# Autodesk Inventor assembly: LowerBody
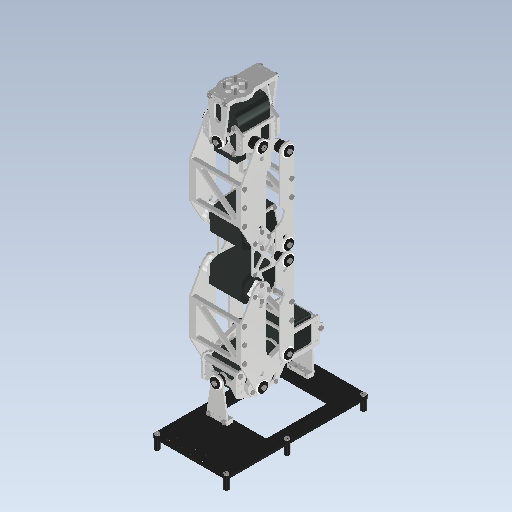
[picture p0: Inventor's stored thumbnail of the model, 512x512]
Saved by Autodesk Inventor 2020.4 (Build 244396010, 396A)
## iProperties
Created: 2021-10-01
Part Number: LowerBody
Document SubType Name: Assembly
Designer: Masato
Mass: 1009.03 g
Surface Area: 2721.67 cm^2
Volume: 456.516 cm^3
Density: 2.21029 g/cm^3
Author: Masato
## Documents named in this file (15)
- C:\Users\t-nagamine\Documents\Cit Brains\OpenPlatform_ver3_0\LowerBody\LowerBody.iam
- C:\Users\t-nagamine\Documents\Cit Brains\OpenPlatform_ver3_0\LowerBody\Ankle\Ankle.iam
- C:\Users\t-nagamine\Documents\Cit Brains\OpenPlatform_ver3_0\LowerBody\Ankle\Ankle_side_pitch.iam
- C:\Users\t-nagamine\Documents\Cit Brains\OpenPlatform_ver3_0\LowerBody\Foot\Foot.iam
- C:\Users\t-nagamine\Documents\Cit Brains\OpenPlatform_ver3_0\LowerBody\Knee\Knee.iam
- C:\Users\t-nagamine\Documents\Cit Brains\OpenPlatform_ver3_0\LowerBody\Leg_joit\Leg_joint_roll_pitch.iam
- C:\Users\t-nagamine\Documents\Cit Brains\OpenPlatform_ver3_0\LowerBody\Leg_joit\Leg_joint_roll_yaw.iam
- C:\Users\t-nagamine\Documents\Cit Brains\OpenPlatform_ver3_0\LowerBody\Slider_crank\Slider_crank_mechanism.iam
- C:\Users\t-nagamine\Documents\Cit Brains\OpenPlatform_ver3_0\LowerBody\Link\BackLink.iam
- C:\Users\t-nagamine\Documents\Cit Brains\OpenPlatform_ver3_0\LowerBody\Link\FrontLink.iam
- C:\Users\t-nagamine\Documents\Cit Brains\OpenPlatform_ver3_0\Ready_Made\Screw\M2_6-6.ipt
- C:\Users\t-nagamine\Documents\Cit Brains\OpenPlatform_ver3_0\Ready_Made\Screw\M3-6.ipt
- C:\Users\t-nagamine\Documents\Cit Brains\OpenPlatform_ver3_0\Ready_Made\Screw\M2_6-10.ipt
- C:\Users\t-nagamine\Documents\Cit Brains\OpenPlatform_ver3_0\Ready_Made\Screw\M3-8.ipt
- C:\Users\t-nagamine\Documents\Cit Brains\OpenPlatform_ver3_0\Ready_Made\Screw\M3-10.ipt
## Components (53 placed, 14 different names)
1. Ankle:1 [sub-assembly] — 挿入:15, 挿入:21, 挿入:22, 角度:11
2. Ankle_side_pitch:1 [sub-assembly] — 挿入:21, 挿入:23, 挿入:24, 挿入:25, 挿入:26, 挿入:35, 挿入:36, フラッシュ:5
3. Ankle_side_pitch:2 [sub-assembly] — 挿入:22, 挿入:27, 挿入:28, 挿入:29, 挿入:30, フラッシュ:5
4. Foot:1 [sub-assembly] — 挿入:15, 挿入:17, 挿入:18, 挿入:19, 挿入:20, 角度:3, 角度:5, 挿入:67
5. Knee:1 [sub-assembly] — 挿入:31, 挿入:32, 挿入:33, 挿入:34
6. Leg_joint_roll_pitch:1 [sub-assembly] — 挿入:2, 挿入:37, 挿入:38, 角度:6, 角度:9, 角度:10, 挿入:70
7. Leg_joint_roll_yaw:1 [sub-assembly] — メイト:1, フラッシュ:3, フラッシュ:4, 角度:5, 角度:6, 挿入:69, 挿入:70
8. Slider_crank_mechanism:1 [sub-assembly] — 挿入:2, 挿入:69
9. BackLink:1 [sub-assembly] — 挿入:33, 挿入:36, 挿入:42, 挿入:46, 挿入:64, 挿入:66, 角度:7
10. FrontLink:1 [sub-assembly] — 挿入:31, 挿入:35, 角度:3, 挿入:51, 挿入:52, 挿入:53, 挿入:54, 挿入:59, 挿入:60, 挿入:61, 挿入:62, 挿入:63, 挿入:65, 角度:7, 角度:11, 角度:12
11. BackLink:2 [sub-assembly] — 挿入:34, 挿入:38, 挿入:39, 挿入:41, 挿入:44, 挿入:45, 角度:8
12. FrontLink:2 [sub-assembly] — 挿入:32, 挿入:37, 挿入:40, 挿入:43, 挿入:47, 挿入:48, 挿入:49, 挿入:50, 挿入:55, 挿入:56, 挿入:57, 挿入:58, 角度:8, 角度:10, 角度:12, 角度:9
13. M2_6-6:9 — 挿入:17
14. M2_6-6:10 — 挿入:18
15. M2_6-6:11 — 挿入:19
16. M2_6-6:12 — 挿入:20
17. M2_6-6:13 — 挿入:23
18. M2_6-6:14 — 挿入:24
19. M2_6-6:15 — 挿入:25
20. M2_6-6:16 — 挿入:26
21. M2_6-6:17 — 挿入:27
22. M2_6-6:18 — 挿入:28
23. M2_6-6:19 — 挿入:29
24. M2_6-6:20 — 挿入:30
25. M3-6:4 — 挿入:40
26. M3-6:5 — 挿入:39
27. M3-6:6 — 挿入:44
28. M3-6:7 — 挿入:43
29. M3-6:8 — 挿入:41
30. M3-6:9 — 挿入:45
31. M3-6:10 — 挿入:42
32. M3-6:11 — 挿入:46
33. M2_6-10:1 — 挿入:47
34. M2_6-10:2 — 挿入:48
35. M2_6-10:3 — 挿入:49
36. M2_6-10:4 — 挿入:50
37. M2_6-10:5 — 挿入:56
38. M2_6-10:6 — 挿入:57
39. M2_6-10:7 — 挿入:58
40. M2_6-10:8 — 挿入:55
41. M2_6-10:9 — 挿入:51
42. M2_6-10:10 — 挿入:52
43. M2_6-10:11 — 挿入:53
44. M2_6-10:12 — 挿入:54
45. M2_6-10:13 — 挿入:59
46. M2_6-10:14 — 挿入:60
47. M2_6-10:15 — 挿入:61
48. M2_6-10:16 — 挿入:62
49. M3-8:1 — 挿入:63
50. M3-8:2 — 挿入:64
51. M3-8:3 — 挿入:66
52. M3-8:4 — 挿入:65
53. M3-10:1 — 挿入:67
## Relationships (68: Insert 55, Angle 9, Flush 3, Mate 1)
- メイト:1 [Mate]: Leg_joint_roll_yaw:1
- フラッシュ:3 [Flush]: Leg_joint_roll_yaw:1
- フラッシュ:4 [Flush]: Leg_joint_roll_yaw:1
- 挿入:2 [Insert]: Leg_joint_roll_pitch:1 ↔ Slider_crank_mechanism:1
- 挿入:15 [Insert]: Ankle:1 ↔ Foot:1
- 挿入:17 [Insert]: Foot:1 ↔ M2_6-6:9
- 挿入:18 [Insert]: Foot:1 ↔ M2_6-6:10
- 挿入:19 [Insert]: Foot:1 ↔ M2_6-6:11
- 挿入:20 [Insert]: Foot:1 ↔ M2_6-6:12
- 挿入:21 [Insert]: Ankle:1 ↔ Ankle_side_pitch:1
- 挿入:22 [Insert]: Ankle:1 ↔ Ankle_side_pitch:2
- 挿入:23 [Insert]: Ankle_side_pitch:1 ↔ M2_6-6:13
- 挿入:24 [Insert]: Ankle_side_pitch:1 ↔ M2_6-6:14
- 挿入:25 [Insert]: Ankle_side_pitch:1 ↔ M2_6-6:15
- 挿入:26 [Insert]: Ankle_side_pitch:1 ↔ M2_6-6:16
- 挿入:27 [Insert]: Ankle_side_pitch:2 ↔ M2_6-6:17
- 挿入:28 [Insert]: Ankle_side_pitch:2 ↔ M2_6-6:18
- 挿入:29 [Insert]: Ankle_side_pitch:2 ↔ M2_6-6:19
- 挿入:30 [Insert]: Ankle_side_pitch:2 ↔ M2_6-6:20
- 挿入:31 [Insert]: Knee:1 ↔ FrontLink:1
- 挿入:32 [Insert]: Knee:1 ↔ FrontLink:2
- 挿入:33 [Insert]: Knee:1 ↔ BackLink:1
- 挿入:34 [Insert]: Knee:1 ↔ BackLink:2
- 挿入:35 [Insert]: Ankle_side_pitch:1 ↔ FrontLink:1
- 挿入:36 [Insert]: Ankle_side_pitch:1 ↔ BackLink:1
- 挿入:37 [Insert]: Leg_joint_roll_pitch:1 ↔ FrontLink:2
- 挿入:38 [Insert]: Leg_joint_roll_pitch:1 ↔ BackLink:2
- 角度:3 [Angle] (0 deg): Foot:1 ↔ FrontLink:1
- 角度:5 [Angle] (0 deg): Foot:1 ↔ Leg_joint_roll_yaw:1
- 挿入:39 [Insert]: BackLink:2 ↔ M3-6:5
- 挿入:40 [Insert]: FrontLink:2 ↔ M3-6:4
- 挿入:41 [Insert]: BackLink:2 ↔ M3-6:8
- 挿入:42 [Insert]: BackLink:1 ↔ M3-6:10
- 挿入:43 [Insert]: FrontLink:2 ↔ M3-6:7
- 挿入:44 [Insert]: BackLink:2 ↔ M3-6:6
- 挿入:45 [Insert]: BackLink:2 ↔ M3-6:9
- 挿入:46 [Insert]: BackLink:1 ↔ M3-6:11
- 挿入:47 [Insert]: FrontLink:2 ↔ M2_6-10:1
- 挿入:48 [Insert]: FrontLink:2 ↔ M2_6-10:2
- 挿入:49 [Insert]: FrontLink:2 ↔ M2_6-10:3
- 挿入:50 [Insert]: FrontLink:2 ↔ M2_6-10:4
- 挿入:51 [Insert]: FrontLink:1 ↔ M2_6-10:9
- 挿入:52 [Insert]: FrontLink:1 ↔ M2_6-10:10
- 挿入:53 [Insert]: FrontLink:1 ↔ M2_6-10:11
- 挿入:54 [Insert]: FrontLink:1 ↔ M2_6-10:12
- 挿入:55 [Insert]: FrontLink:2 ↔ M2_6-10:8
- 挿入:56 [Insert]: FrontLink:2 ↔ M2_6-10:5
- 挿入:57 [Insert]: FrontLink:2 ↔ M2_6-10:6
- 挿入:58 [Insert]: FrontLink:2 ↔ M2_6-10:7
- 挿入:59 [Insert]: FrontLink:1 ↔ M2_6-10:13
- 挿入:60 [Insert]: FrontLink:1 ↔ M2_6-10:14
- 挿入:61 [Insert]: FrontLink:1 ↔ M2_6-10:15
- 挿入:62 [Insert]: FrontLink:1 ↔ M2_6-10:16
- 挿入:63 [Insert]: FrontLink:1 ↔ M3-8:1
- 挿入:64 [Insert]: BackLink:1 ↔ M3-8:2
- 挿入:65 [Insert]: FrontLink:1 ↔ M3-8:4
- 挿入:66 [Insert]: BackLink:1 ↔ M3-8:3
- フラッシュ:5 [Flush]: Ankle_side_pitch:1 ↔ Ankle_side_pitch:2
- 角度:6 [Angle] (0 deg): Leg_joint_roll_pitch:1 ↔ Leg_joint_roll_yaw:1
- 角度:7 [Angle] (0 deg): BackLink:1 ↔ FrontLink:1
- 角度:8 [Angle] (0 deg): BackLink:2 ↔ FrontLink:2
- 挿入:67 [Insert]: Foot:1 ↔ M3-10:1
- 角度:9 [Angle] (0 deg): Leg_joint_roll_pitch:1 ↔ FrontLink:2
- 角度:10 [Angle] (0 deg): Leg_joint_roll_pitch:1 ↔ FrontLink:2
- 角度:11 [Angle] (0 deg): Ankle:1 ↔ FrontLink:1
- 角度:12 [Angle] (0 deg): FrontLink:1 ↔ FrontLink:2
- 挿入:69 [Insert]: Leg_joint_roll_yaw:1 ↔ Slider_crank_mechanism:1
- 挿入:70 [Insert]: Leg_joint_roll_pitch:1 ↔ Leg_joint_roll_yaw:1
